# Autodesk Inventor assembly: robot
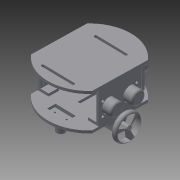
[picture p0: Inventor's stored thumbnail of the model, 180x180]
Saved by Autodesk Inventor 2015 (Build 190159000, 159)
## iProperties
Created: 2014-10-25
Part Number: robot
Document SubType Name: Assembly
Designer: Colin
Author: Colin
## Documents named in this file (6)
- E:\Users\Colin\Documents\college\marc\MicroMouse\robot.iam
- E:\Users\Colin\Documents\college\marc\MicroMouse\base.ipt
- E:\Users\Colin\Documents\college\marc\MicroMouse\wheel_assembly.iam
- E:\Users\Colin\Documents\college\marc\MicroMouse\castor_assembly.iam
- E:\Users\Colin\Documents\college\marc\MicroMouse\ping_assembly.iam
- E:\Users\Colin\Documents\college\marc\MicroMouse\top.ipt
## Components (9 placed, 5 different names)
1. base:1 — Mate:1, Mate:2, Mate:3, Mate:4, Mate:5, Mate:6, Mate:9, Mate:10, Mate:11, Mate:12, Mate:13, Mate:14, Mate:15, Mate:16, Mate:17, Mate:18, Mate:19, Mate:20, Mate:21, Flush:1, Mate:22, Flush:2, Mate:23, Mate:24, Flush:4, Flush:5, Mate:25
2. castor_assembly:1 [sub-assembly] — Mate:1, Mate:2, Mate:3, Mate:15, Mate:16, Mate:17
3. castor_assembly:2 [sub-assembly] — Mate:4, Mate:5, Mate:6, Mate:18, Mate:19, Mate:20
4. wheel_assembly:1 [sub-assembly] — Mate:9, Mate:10, Mate:11
5. wheel_assembly:2 [sub-assembly] — Mate:12, Mate:13, Mate:14
6. ping_assembly:1 [sub-assembly] — Mate:21, Flush:1, Flush:3
7. ping_assembly:2 [sub-assembly] — Mate:22, Flush:2, Mate:23, Flush:3, Flush:6, Mate:26
8. ping_assembly:3 [sub-assembly] — Mate:24, Flush:4, Flush:5
9. top:1 — Mate:25, Flush:6, Mate:26
## Relationships (30: Mate 24, Flush 6)
- Mate:1: base:1 ↔ castor_assembly:1
- Mate:2: base:1 ↔ castor_assembly:1
- Mate:3: base:1 ↔ castor_assembly:1
- Mate:4: base:1 ↔ castor_assembly:2
- Mate:5: base:1 ↔ castor_assembly:2
- Mate:6: base:1 ↔ castor_assembly:2
- Mate:9: base:1 ↔ wheel_assembly:1
- Mate:10: base:1 ↔ wheel_assembly:1
- Mate:11: base:1 ↔ wheel_assembly:1
- Mate:12: base:1 ↔ wheel_assembly:2
- Mate:13: base:1 ↔ wheel_assembly:2
- Mate:14: base:1 ↔ wheel_assembly:2
- Mate:15: base:1 ↔ castor_assembly:1
- Mate:16: base:1 ↔ castor_assembly:1
- Mate:17: base:1 ↔ castor_assembly:1
- Mate:18: base:1 ↔ castor_assembly:2
- Mate:19: base:1 ↔ castor_assembly:2
- Mate:20: base:1 ↔ castor_assembly:2
- Mate:21: base:1 ↔ ping_assembly:1
- Flush:1: base:1 ↔ ping_assembly:1
- Mate:22: base:1 ↔ ping_assembly:2
- Flush:2: base:1 ↔ ping_assembly:2
- Mate:23 (8.1788 mm): base:1 ↔ ping_assembly:2
- Flush:3: ping_assembly:1 ↔ ping_assembly:2
- Mate:24: base:1 ↔ ping_assembly:3
- Flush:4 (12.7 mm): base:1 ↔ ping_assembly:3
- Flush:5: base:1 ↔ ping_assembly:3
- Mate:25: base:1 ↔ top:1
- Flush:6: ping_assembly:2 ↔ top:1
- Mate:26: ping_assembly:2 ↔ top:1
